# Autodesk Inventor assembly: Wózek_inwalidzki
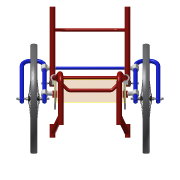
[picture p0: Inventor's stored thumbnail of the model, 180x180]
Saved by Autodesk Inventor 2015 (Build 190159000, 159)
## iProperties
Created: 2016-01-12
Part Number: Wózek_inwalidzki
Document SubType Name: Assembly
Designer: graaapsik
Author: graaapsik
## Documents named in this file (18)
- C:\Users\EriveltonDell\Documents\Centro Universitário da FEI\Wheelchair\CADEIRA DE RODAS - DESENHO\GITHUB\Simplify.iam
- C:\Users\EriveltonDell\Documents\Centro Universitário da FEI\Wheelchair\CADEIRA DE RODAS - DESENHO\lasteverision\Power-Assisted-Wheelchair-master\Koło_tylne.iam
- C:\Users\EriveltonDell\Documents\Centro Universitário da FEI\Wheelchair\CADEIRA DE RODAS - DESENHO\lasteverision\Power-Assisted-Wheelchair-master\Rama_wozka.iam
- C:\Users\EriveltonDell\Documents\Centro Universitário da FEI\Wheelchair\CADEIRA DE RODAS - DESENHO\lasteverision\Power-Assisted-Wheelchair-master\Ciąg.iam
- C:\Users\EriveltonDell\Documents\Centro Universitário da FEI\Wheelchair\CADEIRA DE RODAS - DESENHO\lasteverision\Power-Assisted-Wheelchair-master\GARFO.ipt
- C:\Users\EriveltonDell\Documents\Centro Universitário da FEI\Wheelchair\CADEIRA DE RODAS - DESENHO\lasteverision\Power-Assisted-Wheelchair-master\suporte-rodas-esq.ipt
- C:\Users\EriveltonDell\Documents\Centro Universitário da FEI\Wheelchair\CADEIRA DE RODAS - DESENHO\lasteverision\Power-Assisted-Wheelchair-master\suporte-rodas.ipt
- C:\Users\EriveltonDell\Documents\Centro Universitário da FEI\Wheelchair\CADEIRA DE RODAS - DESENHO\lasteverision\Power-Assisted-Wheelchair-master\suporte-eixo.ipt
- C:\Users\EriveltonDell\Documents\Centro Universitário da FEI\Wheelchair\CADEIRA DE RODAS - DESENHO\lasteverision\Power-Assisted-Wheelchair-master\suporte-barra.ipt
- C:\Users\EriveltonDell\Documents\Centro Universitário da FEI\Wheelchair\CADEIRA DE RODAS - DESENHO\lasteverision\Power-Assisted-Wheelchair-master\Barra-garfo.ipt
- C:\Users\EriveltonDell\Documents\Centro Universitário da FEI\Wheelchair\CADEIRA DE RODAS - DESENHO\lasteverision\Power-Assisted-Wheelchair-master\suporte-eixo - 2.ipt
- C:\Users\EriveltonDell\Documents\Centro Universitário da FEI\Wheelchair\CADEIRA DE RODAS - DESENHO\GITHUB\suporte-barra 2.ipt
- C:\Users\EriveltonDell\Documents\Centro Universitário da FEI\Wheelchair\CADEIRA DE RODAS - DESENHO\lasteverision\Power-Assisted-Wheelchair-master\ISO 4032 - M12ISO.ipt
- C:\Users\EriveltonDell\Documents\Centro Universitário da FEI\Wheelchair\CADEIRA DE RODAS - DESENHO\lasteverision\Power-Assisted-Wheelchair-master\ISO 4032 - M8ISO.ipt
- C:\Users\EriveltonDell\Documents\Centro Universitário da FEI\Wheelchair\CADEIRA DE RODAS - DESENHO\GITHUB\Simplify\AIP\FEA\bvw2lvqww.fins
- C:\Users\EriveltonDell\Documents\Centro Universitário da FEI\Wheelchair\CADEIRA DE RODAS - DESENHO\GITHUB\Simplify\AIP\FEA\bvw2lvqww.fsat
- C:\Users\EriveltonDell\Documents\Centro Universitário da FEI\Wheelchair\CADEIRA DE RODAS - DESENHO\GITHUB\Simplify\AIP\FEA\bvw2lvqww.ftes
- C:\Users\EriveltonDell\Documents\Centro Universitário da FEI\Wheelchair\CADEIRA DE RODAS - DESENHO\GITHUB\Simplify\AIP\FEA\bvw2lvqww.fwiz
## Components (24 placed, 14 different names)
1. Rama_wozka:1 [sub-assembly] — Równoległy:2, Angle:5, 49.15, Insert:13, Insert:14, Angle:12, Angle:13, Angle:14, Mate:63, Tangent:23, Angle:18, Tangent:24, Mate:64
2. Roda [sub-assembly] — Zestawiający:24, Zestawiający:25, Angle:14, Mate:58, Mate:59, Mate:66
3. Koło_tylne:2 [sub-assembly] — Zestawiający:30, Zestawiający:31, Angle:13, Mate:56, Mate:57, Angle:19, Mate:67
4. Ciąg:1 [sub-assembly] — Zestawiający:30, Zestawiający:31
5. Ciąg:2 [sub-assembly] — Zestawiający:24, Zestawiający:25
6. GARFO:1 — Angle:5, Insert:24, Mate:58, Mate:59, Insert:28, Tangent:25, Tangent:27, Tangent:28
7. GARFO:2 — 49.15, Angle:15, Mate:56, Mate:57, Insert:25, Insert:29, Tangent:26, Tangent:29, Tangent:30
8. suporte-rodas-esq:1 — Insert:14, Mate:55, Tangent:19, Tangent:20
9. suporte-rodas:1 — Insert:13, Mate:62, Tangent:21, Tangent:22
10. suporte-eixo:2 — Mate:55, Tangent:19, Tangent:20, Mate:60, Mate:61
11. suporte-barra:1 — Insert:22, Insert:24, Angle:17
12. suporte-barra:2 — Angle:15, Angle:16, Insert:29
13. Barra-garfo:1 — Angle:12, Insert:22
14. suporte-barra:3 — Insert:28, Angle:17, Mate:65
15. suporte-barra:4 — Insert:25, Angle:16, Mate:60, Mate:61
16. suporte-eixo - 2:1 — Mate:62, Tangent:21, Tangent:22, Mate:65
17. suporte-barra 2:1 — Mate:63, Tangent:23, Angle:18, Mate:68, Mate:69
18. suporte-barra 2:2 — Tangent:24, Mate:64, Angle:19, Mate:70, Mate:71
19. ISO 4032 M12:1 — Mate:66, Tangent:25
20. ISO 4032 M12:2 — Mate:67, Tangent:26
21. ISO 4032 M8:1 — Mate:71, Tangent:30
22. ISO 4032 M8:2 — Mate:70, Tangent:29
23. ISO 4032 M8:3 — Mate:69, Tangent:28
24. ISO 4032 M8:4 — Mate:68, Tangent:27
## Relationships (51: Mate 21, Tangent 12, Angle 10, Insert 7, Flush 1)
- Równoległy:2 [Flush]: Rama_wozka:1
- Zestawiający:24 [Mate]: Roda ↔ Ciąg:2
- Zestawiający:25 [Mate]: Roda ↔ Ciąg:2
- Zestawiający:30 [Mate]: Koło_tylne:2 ↔ Ciąg:1
- Zestawiający:31 [Mate]: Koło_tylne:2 ↔ Ciąg:1
- Angle:5 (126 deg): Rama_wozka:1 ↔ GARFO:1
- 49.15 [Angle] (54 deg): Rama_wozka:1 ↔ GARFO:2
- Insert:13 (150 mm): Rama_wozka:1 ↔ suporte-rodas:1
- Insert:14 (150 mm): Rama_wozka:1 ↔ suporte-rodas-esq:1
- Mate:55: suporte-rodas-esq:1 ↔ suporte-eixo:2
- Tangent:19: suporte-rodas-esq:1 ↔ suporte-eixo:2
- Tangent:20: suporte-rodas-esq:1 ↔ suporte-eixo:2
- Angle:12 (0 deg): Rama_wozka:1 ↔ Barra-garfo:1
- Angle:13 (0 deg): Rama_wozka:1 ↔ Koło_tylne:2
- Angle:14 (0 deg): Rama_wozka:1 ↔ Roda
- Insert:22: suporte-barra:1 ↔ Barra-garfo:1
- Angle:15 (0 deg): GARFO:2 ↔ suporte-barra:2
- Mate:56 (10 mm): Koło_tylne:2 ↔ GARFO:2
- Mate:57: Koło_tylne:2 ↔ GARFO:2
- Insert:24: GARFO:1 ↔ suporte-barra:1
- Mate:58: Roda ↔ GARFO:1
- Mate:59 (10 mm): Roda ↔ GARFO:1
- Insert:25 (-100 mm): GARFO:2 ↔ suporte-barra:4
- Angle:16 (0 deg): suporte-barra:2 ↔ suporte-barra:4
- Mate:60: suporte-eixo:2 ↔ suporte-barra:4
- Mate:61: suporte-eixo:2 ↔ suporte-barra:4
- Mate:62: suporte-rodas:1 ↔ suporte-eixo - 2:1
- Insert:28 (-100 mm): GARFO:1 ↔ suporte-barra:3
- Angle:17 (0 deg): suporte-barra:1 ↔ suporte-barra:3
- Insert:29: GARFO:2 ↔ suporte-barra:2
- Tangent:21: suporte-rodas:1 ↔ suporte-eixo - 2:1
- Tangent:22: suporte-rodas:1 ↔ suporte-eixo - 2:1
- Mate:63: Rama_wozka:1 ↔ suporte-barra 2:1
- Tangent:23: Rama_wozka:1 ↔ suporte-barra 2:1
- Angle:18 (0 deg): Rama_wozka:1 ↔ suporte-barra 2:1
- Tangent:24: Rama_wozka:1 ↔ suporte-barra 2:2
- Mate:64: Rama_wozka:1 ↔ suporte-barra 2:2
- Angle:19 (0 deg): Koło_tylne:2 ↔ suporte-barra 2:2
- Mate:65: suporte-barra:3 ↔ suporte-eixo - 2:1
- Mate:66: Roda ↔ ISO 4032 M12:1
- Tangent:25: GARFO:1 ↔ ISO 4032 M12:1
- Mate:67: Koło_tylne:2 ↔ ISO 4032 M12:2
- Tangent:26: GARFO:2 ↔ ISO 4032 M12:2
- Mate:68: suporte-barra 2:1 ↔ ISO 4032 M8:4
- Tangent:27: GARFO:1 ↔ ISO 4032 M8:4
- Mate:69: suporte-barra 2:1 ↔ ISO 4032 M8:3
- Tangent:28: GARFO:1 ↔ ISO 4032 M8:3
- Mate:70: suporte-barra 2:2 ↔ ISO 4032 M8:2
- Tangent:29: GARFO:2 ↔ ISO 4032 M8:2
- Mate:71: suporte-barra 2:2 ↔ ISO 4032 M8:1
- Tangent:30: GARFO:2 ↔ ISO 4032 M8:1
## Named parameters: sa_3 = 950.842, sa_4 = 83.1879, sa_5 = -34987
note: some values were not read from the file. Shown as the stored number, unit unknown: "sa_3", "sa_4", "sa_5".
